# Autodesk Inventor assembly: Cage_connector_v03
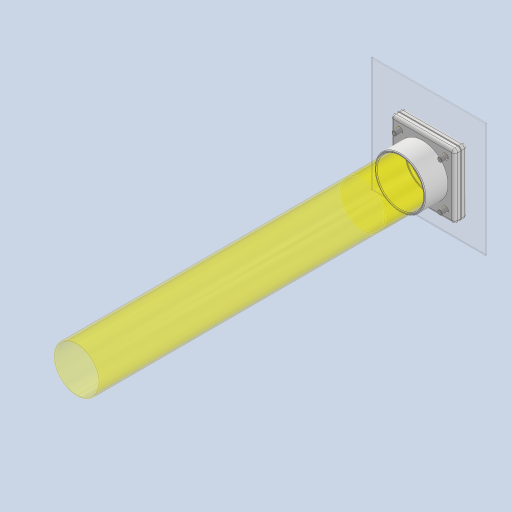
[picture p0: Inventor's stored thumbnail of the model, 512x512]
Saved by Autodesk Inventor 2024.4 (Build 284460000, 460)
## iProperties
Created: 2026-03-25
Part Number: Cage_connector_v03
Document SubType Name: Assembly
Designer: tooles01
Author: tooles01
## iProperties of the stored document MemberDocs/xKrswxfkuLchbobh4Sdohgw0c4c
Created: 2026-03-25
Part Number: Cage_connector_v02
Document SubType Name: Assembly
Designer: tooles01
Author: tooles01
## iProperties of the stored document MemberDocs/xCn5q2qdhM0kstg35Nfetbfz4Yb
Created: 2026-03-25
Part Number: Cage_connector_v02
Document SubType Name: Assembly
Designer: tooles01
Author: tooles01
## iProperties of the stored document MemberDocs/xPbgsdkdlFsqp1bfsCgcvfiahUc
Created: 2026-03-25
Part Number: Cage_connector_v03
Document SubType Name: Assembly
Designer: tooles01
Author: tooles01
## Documents named in this file (8)
- C:\Users\tooles01\NYU Langone Health Dropbox\Shannon Toole\Shannon_Dropbox\Mar lab\RFID\CAD\Cage_connector_v03.iam
- C:\Users\tooles01\NYU Langone Health Dropbox\Shannon Toole\Shannon_Dropbox\Mar lab\RFID\CAD\lib\cage_wall.ipt
- C:\Users\tooles01\NYU Langone Health Dropbox\Shannon Toole\Shannon_Dropbox\Mar lab\RFID\CAD\lib\M3 heat-set insert.ipt
- C:\Users\tooles01\Documents\Inventor\Content Center Files\R2024\en-US\AS 1420\AS 1420 - 1973 - M3 x 10.ipt
- C:\Users\tooles01\NYU Langone Health Dropbox\Shannon Toole\Shannon_Dropbox\Mar lab\RFID\CAD\lib\tube_5cm.ipt
- C:\Users\tooles01\NYU Langone Health Dropbox\Shannon Toole\Shannon_Dropbox\Mar lab\RFID\CAD\lib\tube_25cm.ipt
- C:\Users\tooles01\NYU Langone Health Dropbox\Shannon Toole\Shannon_Dropbox\Mar lab\RFID\CAD\cage_outside_03.ipt
- C:\Users\tooles01\NYU Langone Health Dropbox\Shannon Toole\Shannon_Dropbox\Mar lab\RFID\CAD\cage_inside_03.ipt
## Components (13 placed, 7 different names)
1. cage_wall:1 — cage_inside to wall:1, cage_outside to wall:1
2. cage_inside_03:1 — cage_inside to wall:1, short tube to cage_inside:1, long tube to cage_inside:1, screw to cage_inside:1, screw to cage_inside:2, screw to cage_inside:3, screw to cage_inside:4
3. cage_outside_03:1 — cage_outside to wall:1, heat-set to cage_outside:1, heat-set to cage_outside:2, heat-set to cage_outside:3, heat-set to cage_outside:4
4. tube_5cm:1 — short tube to cage_inside:1
5. tube_25cm:1 — long tube to cage_inside:1
6. M3 heat-set insert:1 — heat-set to cage_outside:1, screw to heat-set:1
7. M3 heat-set insert:2 — heat-set to cage_outside:2, screw to heat-set:2
8. M3 heat-set insert:3 — heat-set to cage_outside:3, screw to heat-set:3
9. M3 heat-set insert:4 — heat-set to cage_outside:4, screw to heat-set:4
10. AS 1420 - Metric M3 x 10:1 — screw to cage_inside:1, screw to heat-set:1
11. AS 1420 - Metric M3 x 10:2 — screw to cage_inside:2, screw to heat-set:2
12. AS 1420 - Metric M3 x 10:3 — screw to cage_inside:3, screw to heat-set:3
13. AS 1420 - Metric M3 x 10:4 — screw to cage_inside:4, screw to heat-set:4
## Relationships (16: Insert 12, Mate 4)
- cage_inside to wall:1 [Insert]: cage_wall:1 ↔ cage_inside_03:1
- cage_outside to wall:1 [Insert]: cage_wall:1 ↔ cage_outside_03:1
- short tube to cage_inside:1 [Insert]: cage_inside_03:1 ↔ tube_5cm:1
- long tube to cage_inside:1 [Insert]: cage_inside_03:1 ↔ tube_25cm:1
- heat-set to cage_outside:1 [Insert]: cage_outside_03:1 ↔ M3 heat-set insert:1
- heat-set to cage_outside:2 [Insert]: cage_outside_03:1 ↔ M3 heat-set insert:2
- heat-set to cage_outside:3 [Insert]: cage_outside_03:1 ↔ M3 heat-set insert:3
- heat-set to cage_outside:4 [Insert]: cage_outside_03:1 ↔ M3 heat-set insert:4
- screw to cage_inside:1 [Insert]: cage_inside_03:1 ↔ AS 1420 - Metric M3 x 10:1
- screw to cage_inside:2 [Insert]: cage_inside_03:1 ↔ AS 1420 - Metric M3 x 10:2
- screw to cage_inside:3 [Insert]: cage_inside_03:1 ↔ AS 1420 - Metric M3 x 10:3
- screw to cage_inside:4 [Insert]: cage_inside_03:1 ↔ AS 1420 - Metric M3 x 10:4
- screw to heat-set:1 [Mate]: M3 heat-set insert:1 ↔ AS 1420 - Metric M3 x 10:1
- screw to heat-set:2 [Mate]: M3 heat-set insert:2 ↔ AS 1420 - Metric M3 x 10:2
- screw to heat-set:3 [Mate]: M3 heat-set insert:3 ↔ AS 1420 - Metric M3 x 10:3
- screw to heat-set:4 [Mate]: M3 heat-set insert:4 ↔ AS 1420 - Metric M3 x 10:4
